# Autodesk Inventor assembly: Turret Assembly
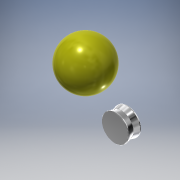
[picture p0: Inventor's stored thumbnail of the model, 180x180]
Saved by Autodesk Inventor 2019.4 (Build 234330000, 330)
## iProperties
Created: 2020-01-16
Part Number: Turret Assembly
Document SubType Name: Assembly
Designer: admin
Author: admin
## Documents named in this file (3)
- C:\Users\admin\Desktop\FRC 2020 Engineering\GitHub\7738-2020\Robot V2\Turret\Turret Assembly.iam
- C:\Users\admin\Desktop\FRC 2020 Engineering\GitHub\7738-2020\Robot V2\Turret\Flywheel Half.ipt
- C:\Users\admin\Desktop\FRC 2020 Engineering\GitHub\7738-2020\Power Cell.ipt
## Components (3 placed, 2 different names)
1. Flywheel Half:1 — Mate:1, Mate:2
2. Flywheel Half:2 — Mate:1, Mate:2
3. Power Cell:1
## Relationships (2: Mate 2)
- Mate:1: Flywheel Half:1 ↔ Flywheel Half:2
- Mate:2: Flywheel Half:1 ↔ Flywheel Half:2
